# Autodesk Inventor assembly: L_Unit_SR-T
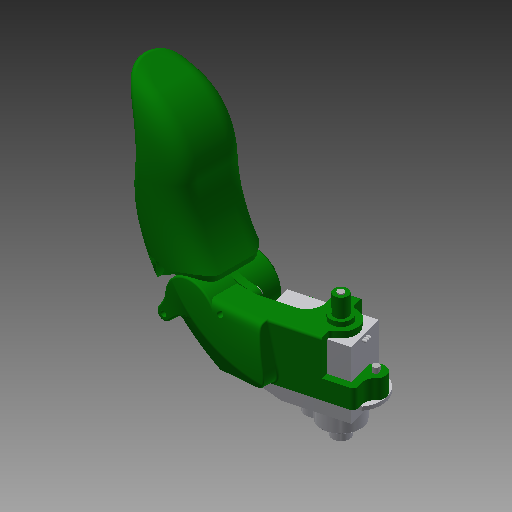
[picture p0: Inventor's stored thumbnail of the model, 512x512]
Saved by Autodesk Inventor 2018.3 (Build 223284000, 284)
## iProperties
Created: 2018-02-15
Part Number: L_Unit_SR-T
Material: 一般
Document SubType Name: Assembly
Designer: sktom
Title: Unit_SR-T
Author: sktom
## Documents named in this file (10)
- D:\CloudStrage\OneDrive\CADMech\HbSizeSMech\UnitHand\Unit_SR-H\Unit_SR-T\L_Unit_SR-T.iam
- D:\CloudStrage\OneDrive\CADMech\HbSizeSMech\UnitHand\Unit_SR-H\Unit_SR-T\L_SR-T-01.ipt
- D:\CloudStrage\OneDrive\CADMech\HbSizeSMech\UnitHand\Unit_SR-H\Unit_SR-T\L_SR-T-02.ipt
- D:\CloudStrage\OneDrive\CADMech\HbSizeSMech\UnitHand\Unit_SR-H\Unit_SR-T\L_SR-T-03.ipt
- D:\CloudStrage\OneDrive\CADMech\HbSizeSMech\UnitHand\Unit_SR-H\Unit_SR-T\L_SR-T-04.ipt
- D:\CloudStrage\OneDrive\CADMech\HbSizeSMech\UnitHand\Unit_SR-H\Unit_SR-T\L_SR-T-05.ipt
- D:\CloudStrage\OneDrive\CADMech\HbSizeSMech\UnitHand\Unit_SR-H\Unit_SR-T\L_SR-T-06.ipt
- D:\CloudStrage\OneDrive\CADMech\HbSizeSMech\UnitHand\Unit_SR-H\Unit_SR-T\L_Parts_Servo_HK282A.ipt
- D:\CloudStrage\OneDrive\CADMech\HbSizeSMech\UnitHand\Unit_SR-H\Unit_SR-T\L_Parts_CoilSpring_CP 0.5-4.5-6.5.ipt
- D:\CloudStrage\OneDrive\CADMech\HbSizeSMech\UnitHand\Unit_SR-H\Unit_SR-T\L_Parts_Screw_M1.4_L6.ipt
## Components (14 placed, 9 different names)
1. L_SR-T-01:1 — 挿入:5, 挿入:9
2. L_SR-T-02:1 — 挿入:4, 挿入:5
3. L_SR-T-03:1 — 挿入:3, 挿入:4, 挿入:2, 挿入:1, 挿入:7, 挿入:6, 挿入:14, 挿入:15
4. L_SR-T-04:1 — 挿入:3
5. L_SR-T-05:1 — 挿入:2, 挿入:1, 挿入:10, 挿入:11
6. L_SR-T-06:1 — 挿入:8, 挿入:12
7. L_Parts_Servo_HK282A:1 — 挿入:7, 挿入:6, 挿入:8, 挿入:13
8. L_Parts_CoilSpring_CP 0.5-4.5-6.5:1 — 挿入:15
9. L_Parts_Screw_M1.4_L6:1 — 挿入:9
10. L_Parts_Screw_M1.4_L6:2 — 挿入:10
11. L_Parts_Screw_M1.4_L6:3 — 挿入:11
12. L_Parts_Screw_M1.4_L6:4 — 挿入:12
13. L_Parts_Screw_M1.4_L6:5 — 挿入:13
14. L_Parts_Screw_M1.4_L6:6 — 挿入:14
## Relationships (15: Insert 15)
- 挿入:3 [Insert] (1 mm): L_SR-T-03:1 ↔ L_SR-T-04:1
- 挿入:4 [Insert] (0.1 mm): L_SR-T-02:1 ↔ L_SR-T-03:1
- 挿入:2 [Insert]: L_SR-T-03:1 ↔ L_SR-T-05:1
- 挿入:1 [Insert]: L_SR-T-03:1 ↔ L_SR-T-05:1
- 挿入:5 [Insert]: L_SR-T-01:1 ↔ L_SR-T-02:1
- 挿入:7 [Insert]: L_SR-T-03:1 ↔ L_Parts_Servo_HK282A:1
- 挿入:6 [Insert]: L_SR-T-03:1 ↔ L_Parts_Servo_HK282A:1
- 挿入:8 [Insert]: L_SR-T-06:1 ↔ L_Parts_Servo_HK282A:1
- 挿入:9 [Insert]: L_SR-T-01:1 ↔ L_Parts_Screw_M1.4_L6:1
- 挿入:10 [Insert]: L_SR-T-05:1 ↔ L_Parts_Screw_M1.4_L6:2
- 挿入:11 [Insert]: L_SR-T-05:1 ↔ L_Parts_Screw_M1.4_L6:3
- 挿入:12 [Insert]: L_SR-T-06:1 ↔ L_Parts_Screw_M1.4_L6:4
- 挿入:13 [Insert]: L_Parts_Servo_HK282A:1 ↔ L_Parts_Screw_M1.4_L6:5
- 挿入:14 [Insert]: L_SR-T-03:1 ↔ L_Parts_Screw_M1.4_L6:6
- 挿入:15 [Insert]: L_SR-T-03:1 ↔ L_Parts_CoilSpring_CP 0.5-4.5-6.5:1
